# Autodesk Inventor assembly: hoops_sml_med_lrg
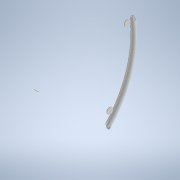
[picture p0: Inventor's stored thumbnail of the model, 180x180]
Saved by Autodesk Inventor 2021 (Build 250183000, 183)
## iProperties
Created: 2021-05-05
Part Number: hoops_sml_med_lrg
Document SubType Name: Assembly
## Documents named in this file (10)
- C:\Users\ocon0143\OneDrive - Flinders\Advn Mech Design Shared\6_Development\2_Design\inventor\hoop_slider\hoops_sml_med_lrg.iam
- C:\Users\ocon0143\OneDrive - Flinders\Advn Mech Design Shared\6_Development\2_Design\inventor\hoop_slider\large_hoop.ipt
- C:\Users\ocon0143\OneDrive - Flinders\Advn Mech Design Shared\6_Development\2_Design\inventor\hoop_slider\medium_hoop.ipt
- C:\Users\ocon0143\OneDrive - Flinders\Advn Mech Design Shared\6_Development\2_Design\inventor\rack_pinion\pinion.ipt
- C:\Users\ocon0143\OneDrive - Flinders\Advn Mech Design Shared\6_Development\2_Design\inventor\hoop_slider\small_hoop.ipt
- C:\Users\ocon0143\OneDrive - Flinders\Advn Mech Design Shared\6_Development\2_Design\inventor\rack_pinion\tooth.ipt
- C:\Users\ocon0143\OneDrive - Flinders\Advn Mech Design Shared\6_Development\2_Design\inventor\rack_pinion\pulley_guide.ipt
- C:\Users\ocon0143\OneDrive - Flinders\Advn Mech Design Shared\6_Development\2_Design\inventor\rack_pinion\large_bearings.ipt
- C:\Users\ocon0143\OneDrive - Flinders\Advn Mech Design Shared\6_Development\2_Design\inventor\rack_pinion\medium_bearings.ipt
- C:\Users\ocon0143\OneDrive - Flinders\Advn Mech Design Shared\6_Development\2_Design\inventor\params.xlsx
## Components (68 placed, 8 different names)
1. large_hoop:1 — Mate:1, Flush:1, Flush:12
2. medium_hoop:1 — Mate:2, Flush:2, Mate:4, Flush:8, Flush:9, Mate:6, Mate:7
3. pinion:1 — Flush:6
4. small_hoop:1 — Mate:3, Flush:7, Mate:8, Mate:9
5. large_bearings:1 — Mate:6, Flush:12
6. medium_bearings:1 — Flush:13, Mate:7
7. pinion:2
8. pulley_guide:1 — Mate:8, Mate:9, Mate:10
9. tooth:1 — Mate:4, Flush:8, Flush:9
10. tooth:2
11. tooth:3
12. tooth:4
13. tooth:5
14. tooth:6
15. tooth:7
16. tooth:8
17. tooth:9
18. tooth:10
19. tooth:11
20. tooth:12
21. tooth:13
22. tooth:14
23. tooth:15
24. tooth:16
25. tooth:17
26. tooth:18
27. tooth:19
28. tooth:20
29. tooth:21
30. tooth:22
31. tooth:23
32. tooth:24
33. tooth:25
34. tooth:26
35. tooth:27
36. tooth:28
37. tooth:29
38. tooth:30
39. tooth:31
40. tooth:32
41. tooth:33
42. tooth:34
43. tooth:35
44. tooth:36
45. tooth:37
46. tooth:38
47. tooth:39
48. tooth:40
49. tooth:41
50. tooth:42
51. tooth:43
52. tooth:44
53. tooth:45
54. tooth:46
55. tooth:47
56. tooth:48
57. tooth:49
58. tooth:50
59. tooth:51
60. tooth:52
61. tooth:53
62. tooth:54
63. tooth:55
64. tooth:56
65. tooth:57
66. tooth:58
67. tooth:59
68. tooth:60
## Component patterns: (60 elements, first: tooth:1)
## Relationships (17: Mate 9, Flush 8)
- Mate:1: large_hoop:1
- Mate:2: medium_hoop:1
- Flush:1: large_hoop:1
- Flush:2: medium_hoop:1
- Flush:6: pinion:1
- Mate:3: small_hoop:1
- Flush:7: small_hoop:1
- Mate:4: medium_hoop:1 ↔ tooth:1
- Flush:8: medium_hoop:1 ↔ tooth:1
- Flush:9: medium_hoop:1 ↔ tooth:1
- Mate:6: medium_hoop:1 ↔ large_bearings:1
- Flush:12: large_hoop:1 ↔ large_bearings:1
- Flush:13: medium_bearings:1
- Mate:7: medium_hoop:1 ↔ medium_bearings:1
- Mate:8 (-10 mm): small_hoop:1 ↔ pulley_guide:1
- Mate:9: small_hoop:1 ↔ pulley_guide:1
- Mate:10: pulley_guide:1
## Named parameters: testLength = 1700 mm, testWidth = 1500 mm, testHeight = 1000 mm, rack_tooth_thickness = 5 mm, rack_tooth_face_widh = 10 mm, rack_tooth_addendum = 5 mm, rack_tooth_dedendum = 5 mm, hoop_radius_large = 3300 mm, hoop_width_large = 80 mm, hoop_thickness_large = 10 mm, hoop_width_medium = 60 mm, hoop_thickness_medium = 10 mm, hoop_width_small = 40 mm, hoop_thickness_small = 10 mm, hoop_height_large = 450 mm, hoop_height_medium = 450 mm, hoop_height_small = 600 mm, hoop_length_large = 200 mm, hoop_length_medium = 700 mm, hoop_length_small = 700 mm, cover_width_main = 1400 mm, cover_height_main = 600 mm, cover_length_main = 1600 mm, cover_shell_thickness = 10 mm, cover_base_thickness = 10 mm, cover_mountHole_diameter = 10 mm, cover_mountHole_xSpacing = 900 mm, cover_mountHole_ySpacing = 550 mm, cover_side_thickness = 20 mm, cover_side_openSize = 1000 mm, hoop_bearing_length = 5 deg, hoop_cable_diam = 5 mm, hoop_cable_pulley_diam = 22 mm, secure_arm_length = 400 mm, secure_arm_radii = 9 mm, secure_arm_hold_length = 35 mm, secure_arm_hold_thickness = 10 mm, secure_arm_thickness = 20 mm, secure_arm_angle = 20 deg
